# Autodesk Inventor assembly: Assy_all_body
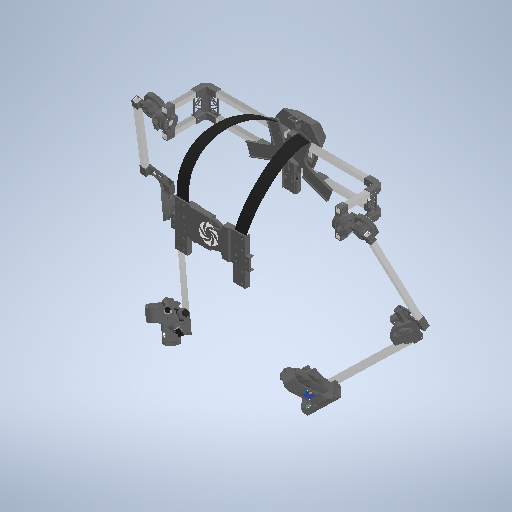
[picture p0: Inventor's stored thumbnail of the model, 512x512]
Saved by Autodesk Inventor 2026.1 (Build 301233020, 233B)
## iProperties
Created: 2026-02-03
Part Number: Assy_all_body
Document SubType Name: Assembly
Designer: hibik
Author: hibik
## Documents named in this file (5)
- C:\Users\hibik\Documents\Robomech\HR\controller\hard\Assy_all_body.iam
- C:\Users\hibik\Documents\Robomech\HR\controller\hard\body\Assy_body.iam
- C:\Users\hibik\Documents\Robomech\HR\controller\hard\body\pole_setter_handle.ipt
- C:\Users\hibik\Documents\Robomech\HR\controller\hard\handle_right\handle.iam
- C:\Users\hibik\Documents\Robomech\HR\controller\hard\handle_left\handle_left.iam
## Components (5 placed, 4 different names)
1. Assy_body:1 [sub-assembly] — 挿入:1, 角度:1, 挿入:2, 角度:2
2. pole_setter_handle:1 — 挿入:1, 角度:1, 挿入:3, 角度:3
3. pole_setter_handle:2 — 挿入:2, 角度:2, 挿入:4, 角度:4
4. handle:1 [sub-assembly] — 挿入:3, 角度:3
5. handle_left:1 [sub-assembly] — 挿入:4, 角度:4
## Relationships (8: Insert 4, Angle 4)
- 挿入:1 [Insert]: Assy_body:1 ↔ pole_setter_handle:1
- 角度:1 [Angle] (0 deg): Assy_body:1 ↔ pole_setter_handle:1
- 挿入:2 [Insert]: Assy_body:1 ↔ pole_setter_handle:2
- 角度:2 [Angle] (0 deg): Assy_body:1 ↔ pole_setter_handle:2
- 挿入:3 [Insert]: pole_setter_handle:1 ↔ handle:1
- 角度:3 [Angle] (0 deg): pole_setter_handle:1 ↔ handle:1
- 挿入:4 [Insert]: pole_setter_handle:2 ↔ handle_left:1
- 角度:4 [Angle] (0 deg): pole_setter_handle:2 ↔ handle_left:1
